# Autodesk Inventor assembly: body
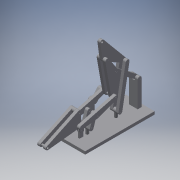
[picture p0: Inventor's stored thumbnail of the model, 180x180]
Saved by Autodesk Inventor 2016 (Build 200138000, 138)
## iProperties
Created: 2018-05-06
Part Number: body
Material: 一般
Document SubType Name: Assembly
Designer: 黃胤瑋
Author: 黃胤瑋
## Documents named in this file (20)
- C:\Users\黃胤瑋\Desktop\mechanism\Two stage six link lifting mechanism\body.iam
- C:\Users\黃胤瑋\Desktop\mechanism\Two stage six link lifting mechanism\實體1.ipt
- C:\Users\黃胤瑋\Desktop\mechanism\Two stage six link lifting mechanism\實體2.ipt
- C:\Users\黃胤瑋\Desktop\mechanism\Two stage six link lifting mechanism\實體3.ipt
- C:\Users\黃胤瑋\Desktop\mechanism\Two stage six link lifting mechanism\實體4.ipt
- C:\Users\黃胤瑋\Desktop\mechanism\Two stage six link lifting mechanism\實體5.ipt
- C:\Users\黃胤瑋\Desktop\mechanism\Two stage six link lifting mechanism\實體6.ipt
- C:\Users\黃胤瑋\Desktop\mechanism\Two stage six link lifting mechanism\實體7.ipt
- C:\Users\黃胤瑋\Desktop\mechanism\Two stage six link lifting mechanism\實體9.ipt
- C:\Users\黃胤瑋\Desktop\mechanism\Two stage six link lifting mechanism\實體10.ipt
- C:\Users\黃胤瑋\Desktop\mechanism\Two stage six link lifting mechanism\實體11.ipt
- C:\Users\黃胤瑋\Desktop\mechanism\Two stage six link lifting mechanism\實體12.ipt
- C:\Users\黃胤瑋\Desktop\mechanism\Two stage six link lifting mechanism\實體13.ipt
- C:\Users\黃胤瑋\Desktop\mechanism\Two stage six link lifting mechanism\實體14.ipt
- C:\Users\黃胤瑋\Desktop\mechanism\Two stage six link lifting mechanism\實體15.ipt
- C:\Users\黃胤瑋\Desktop\mechanism\Two stage six link lifting mechanism\實體16.ipt
- C:\Users\黃胤瑋\Desktop\mechanism\Two stage six link lifting mechanism\銷6.ipt
- C:\Users\黃胤瑋\Desktop\mechanism\Two stage six link lifting mechanism\銷9.ipt
- C:\Users\黃胤瑋\Desktop\mechanism\Two stage six link lifting mechanism\銷12.ipt
- C:\Users\黃胤瑋\Desktop\mechanism\Two stage six link lifting mechanism\銷3.ipt
## Components (30 placed, 19 different names)
1. 實體1:1 — 貼合:41, 貼合:47, 貼合:50, 貼合:51
2. 實體2:1 — 貼合:44, 貼合:45, 貼合:46, 角度:1, 貼合:73, 齊平:21
3. 實體3:1 — 貼合:57, 貼合:58, 貼合:59
4. 實體4:1 — 貼合:54, 貼合:56, 貼合:61, 貼合:64
5. 實體5:1 — 貼合:12, 齊平:8, 貼合:13, 齊平:9, 貼合:43, 貼合:49, 貼合:52, 貼合:59
6. 實體6:1 — 貼合:48, 貼合:49, 貼合:51, 貼合:53, 貼合:55, 貼合:56
7. 實體7:1 — 貼合:14, 齊平:10, 貼合:16, 齊平:12, 貼合:55
8. 實體9:1 — 貼合:7, 齊平:7, 貼合:20, 貼合:23, 貼合:69, 齊平:18
9. 實體10:1 — 貼合:2, 貼合:34, 貼合:36, 貼合:39, 貼合:71, 齊平:19
10. 實體11:1 — 齊平:3, 貼合:27, 貼合:29, 貼合:34, 貼合:35, 貼合:37
11. 實體12:1 — 齊平:2, 貼合:3, 貼合:30, 貼合:32, 貼合:33, 貼合:36, 貼合:38
12. 實體13:1 — 貼合:17, 齊平:13, 貼合:27, 貼合:28, 齊平:15, 貼合:63, 貼合:68
13. 實體14:1 — 貼合:23, 貼合:31, 貼合:42, 貼合:43, 貼合:52, 貼合:70
14. 實體15:1 — 貼合:63, 貼合:65, 貼合:67, 齊平:17
15. 實體16:1 — 貼合:15, 齊平:11, 貼合:19, 貼合:20, 貼合:39, 貼合:44, 貼合:46, 貼合:58, 貼合:60, 貼合:61, 角度:1, 貼合:72, 齊平:20
16. 銷6:1 — 貼合:3, 齊平:3, 貼合:32, 貼合:37, 貼合:38
17. 銷9:1 — 貼合:2, 齊平:2, 貼合:33, 貼合:35
18. 銷9:4 — 貼合:13, 齊平:9, 貼合:47, 貼合:48, 貼合:50
19. 銷9:6 — 貼合:12, 齊平:8
20. 銷9:7 — 貼合:7, 齊平:7, 貼合:19, 貼合:65
21. 銷9:9 — 貼合:14, 齊平:10, 貼合:53, 貼合:54
22. 銷9:10 — 貼合:15, 齊平:11, 貼合:57
23. 銷9:11 — 貼合:16, 齊平:12, 貼合:60, 貼合:64
24. 銷12:6 — 貼合:17, 齊平:13, 貼合:41, 貼合:42, 貼合:45
25. 銷12:8 — 貼合:28, 齊平:15, 貼合:29, 貼合:30, 貼合:31
26. 銷6:3 — 貼合:67, 貼合:68, 齊平:17
27. 銷6:4 — 貼合:69, 貼合:70, 齊平:18
28. 銷3:1 — 貼合:71, 齊平:19
29. 銷6:5 — 貼合:72, 齊平:20
30. 銷3:2 — 貼合:73, 齊平:21
## Relationships (72: Mate 56, Flush 15, Angle 1)
- 貼合:2 [Mate]: 實體10:1 ↔ 銷9:1
- 齊平:2 [Flush]: 實體12:1 ↔ 銷9:1
- 貼合:3 [Mate]: 實體12:1 ↔ 銷6:1
- 齊平:3 [Flush]: 實體11:1 ↔ 銷6:1
- 貼合:7 [Mate]: 實體9:1 ↔ 銷9:7
- 齊平:7 [Flush]: 實體9:1 ↔ 銷9:7
- 貼合:12 [Mate]: 實體5:1 ↔ 銷9:6
- 齊平:8 [Flush]: 實體5:1 ↔ 銷9:6
- 貼合:13 [Mate]: 實體5:1 ↔ 銷9:4
- 齊平:9 [Flush]: 實體5:1 ↔ 銷9:4
- 貼合:14 [Mate]: 實體7:1 ↔ 銷9:9
- 齊平:10 [Flush]: 實體7:1 ↔ 銷9:9
- 貼合:15 [Mate]: 實體16:1 ↔ 銷9:10
- 齊平:11 [Flush]: 實體16:1 ↔ 銷9:10
- 貼合:16 [Mate]: 實體7:1 ↔ 銷9:11
- 齊平:12 [Flush]: 實體7:1 ↔ 銷9:11
- 貼合:17 [Mate]: 實體13:1 ↔ 銷12:6
- 齊平:13 [Flush]: 實體13:1 ↔ 銷12:6
- 貼合:19 [Mate]: 實體16:1 ↔ 銷9:7
- 貼合:20 [Mate]: 實體9:1 ↔ 實體16:1
- 貼合:23 [Mate]: 實體9:1 ↔ 實體14:1
- 貼合:27 [Mate]: 實體11:1 ↔ 實體13:1
- 貼合:28 [Mate]: 實體13:1 ↔ 銷12:8
- 齊平:15 [Flush]: 實體13:1 ↔ 銷12:8
- 貼合:29 [Mate]: 實體11:1 ↔ 銷12:8
- 貼合:30 [Mate]: 實體12:1 ↔ 銷12:8
- 貼合:31 [Mate]: 實體14:1 ↔ 銷12:8
- 貼合:32 [Mate]: 實體12:1 ↔ 銷6:1
- 貼合:33 [Mate]: 實體12:1 ↔ 銷9:1
- 貼合:34 [Mate]: 實體10:1 ↔ 實體11:1
- 貼合:35 [Mate]: 實體11:1 ↔ 銷9:1
- 貼合:36 [Mate]: 實體10:1 ↔ 實體12:1
- 貼合:37 [Mate]: 實體11:1 ↔ 銷6:1
- 貼合:38 [Mate]: 實體12:1 ↔ 銷6:1
- 貼合:39 [Mate]: 實體10:1 ↔ 實體16:1
- 貼合:41 [Mate]: 實體1:1 ↔ 銷12:6
- 貼合:42 [Mate]: 實體14:1 ↔ 銷12:6
- 貼合:43 [Mate]: 實體5:1 ↔ 實體14:1
- 貼合:44 [Mate]: 實體2:1 ↔ 實體16:1
- 貼合:45 [Mate]: 實體2:1 ↔ 銷12:6
- 貼合:46 [Mate]: 實體2:1 ↔ 實體16:1
- 貼合:47 [Mate]: 實體1:1 ↔ 銷9:4
- 貼合:48 [Mate]: 實體6:1 ↔ 銷9:4
- 貼合:49 [Mate]: 實體5:1 ↔ 實體6:1
- 貼合:50 [Mate]: 實體1:1 ↔ 銷9:4
- 貼合:51 [Mate]: 實體1:1 ↔ 實體6:1
- 貼合:52 [Mate]: 實體5:1 ↔ 實體14:1
- 貼合:53 [Mate]: 實體6:1 ↔ 銷9:9
- 貼合:54 [Mate]: 實體4:1 ↔ 銷9:9
- 貼合:55 [Mate]: 實體6:1 ↔ 實體7:1
- 貼合:56 [Mate]: 實體4:1 ↔ 實體6:1
- 貼合:57 [Mate]: 實體3:1 ↔ 銷9:10
- 貼合:58 [Mate]: 實體3:1 ↔ 實體16:1
- 貼合:59 [Mate]: 實體3:1 ↔ 實體5:1
- 貼合:60 [Mate]: 實體16:1 ↔ 銷9:11
- 貼合:61 [Mate]: 實體4:1 ↔ 實體16:1
- 貼合:63 [Mate]: 實體13:1 ↔ 實體15:1
- 角度:1 [Angle] (1042 deg): 實體2:1 ↔ 實體16:1
- 貼合:64 [Mate]: 實體4:1 ↔ 銷9:11
- 貼合:65 [Mate]: 實體15:1 ↔ 銷9:7
- 貼合:67 [Mate]: 實體15:1 ↔ 銷6:3
- 貼合:68 [Mate]: 實體13:1 ↔ 銷6:3
- 齊平:17 [Flush]: 實體15:1 ↔ 銷6:3
- 貼合:69 [Mate]: 實體9:1 ↔ 銷6:4
- 貼合:70 [Mate]: 實體14:1 ↔ 銷6:4
- 齊平:18 [Flush]: 實體9:1 ↔ 銷6:4
- 貼合:71 [Mate]: 實體10:1 ↔ 銷3:1
- 齊平:19 [Flush]: 實體10:1 ↔ 銷3:1
- 貼合:72 [Mate]: 實體16:1 ↔ 銷6:5
- 齊平:20 [Flush]: 實體16:1 ↔ 銷6:5
- 貼合:73 [Mate]: 實體2:1 ↔ 銷3:2
- 齊平:21 [Flush]: 實體2:1 ↔ 銷3:2
